# Autodesk Inventor assembly: Сборка1
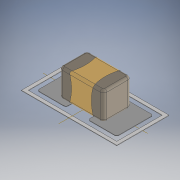
[picture p0: Inventor's stored thumbnail of the model, 180x180]
Saved by Autodesk Inventor 2022 (Build 260153000, 153)
## iProperties
Created: 2022-12-24
Part Number: Сборка1
Document SubType Name: Assembly
Designer: Ivan Petrov
Author: Ivan Petrov
## Documents named in this file (2)
- C:\Users\Ivan Petrov\Documents\GitHub\OmniBot\design\standart_components\Capacitors smd\Сборка1.iam
- C:\Users\Ivan Petrov\Documents\GitHub\OmniBot\design\standart_components\Capacitors smd\C0805.ipt
## Components (1 placed, 1 different names)
1. C0805:1 — Совмещение:1, Совмещение:2, Совмещение:4, Совмещение:5, Угол:1
## Relationships (7: Mate 6, Angle 1)
- Совмещение:1 [Mate]: C0805:1
- Совмещение:2 [Mate]: C0805:1
- Совмещение:3 [Mate]
- Совмещение:4 [Mate]: C0805:1
- Совмещение:5 [Mate]: C0805:1
- Совмещение:6 [Mate]
- Угол:1 [Angle] (-90 deg): C0805:1
